# Autodesk Inventor assembly: spoolHolder
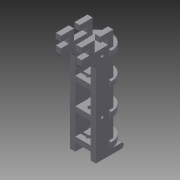
[picture p0: Inventor's stored thumbnail of the model, 180x180]
Saved by Autodesk Inventor 2013 (Build 170138000, 138)
## iProperties
Created: 2015-01-14
Part Number: spoolHolder
Document SubType Name: Assembly
Designer: dzban
Author: dzban
## Documents named in this file (4)
- D:\PIRX\Artisan\OPENSOURCE\SmallPieces\spoolHolder.iam
- D:\PIRX\Artisan\OPENSOURCE\SmallPieces\spoolHolder_c.ipt
- D:\PIRX\Artisan\OPENSOURCE\SmallPieces\spoolHolder_a.ipt
- D:\PIRX\Artisan\OPENSOURCE\SmallPieces\spoolHolder_b.ipt
## Components (6 placed, 3 different names)
1. spoolHolder_c:1 — Mate:1, Mate:6, Mate:11
2. spoolHolder_a:1 — Mate:1, Mate:2, Mate:3, Mate:4, Flush:1, Flush:2, Mate:6, Mate:7, Mate:8, Mate:9, Mate:11, Mate:13
3. spoolHolder_b:1 — Mate:5, Flush:1, Flush:2, Mate:10, Mate:12
4. spoolHolder_c:2 — Mate:3, Mate:8, Mate:12
5. spoolHolder_c:3 — Mate:4, Mate:9, Mate:10
6. spoolHolder_c:4 — Mate:2, Mate:5, Mate:7, Mate:13
## Relationships (15: Mate 13, Flush 2)
- Mate:1: spoolHolder_c:1 ↔ spoolHolder_a:1
- Mate:2: spoolHolder_a:1 ↔ spoolHolder_c:4
- Mate:3: spoolHolder_a:1 ↔ spoolHolder_c:2
- Mate:4: spoolHolder_a:1 ↔ spoolHolder_c:3
- Mate:5: spoolHolder_b:1 ↔ spoolHolder_c:4
- Flush:1: spoolHolder_a:1 ↔ spoolHolder_b:1
- Flush:2: spoolHolder_a:1 ↔ spoolHolder_b:1
- Mate:6: spoolHolder_c:1 ↔ spoolHolder_a:1
- Mate:7: spoolHolder_a:1 ↔ spoolHolder_c:4
- Mate:8: spoolHolder_a:1 ↔ spoolHolder_c:2
- Mate:9: spoolHolder_a:1 ↔ spoolHolder_c:3
- Mate:10: spoolHolder_b:1 ↔ spoolHolder_c:3
- Mate:11: spoolHolder_c:1 ↔ spoolHolder_a:1
- Mate:12: spoolHolder_b:1 ↔ spoolHolder_c:2
- Mate:13: spoolHolder_a:1 ↔ spoolHolder_c:4
